# Autodesk Inventor assembly: one_servo_test
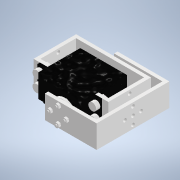
[picture p0: Inventor's stored thumbnail of the model, 180x180]
Saved by Autodesk Inventor 2021.4 (Build 254397000, 397)
## iProperties
Created: 2022-07-24
Part Number: one_servo_test
Document SubType Name: Assembly
Designer: isamu
Author: isamu
## Documents named in this file (3)
- D:\personal_projects\robot\inventor\2021_export_exp\one_servo_test.iam
- D:\personal_projects\robot\inventor\2021_export_exp\mg996r_rot_frame.iam
- D:\personal_projects\robot\inventor\2021_export_exp\mg996r_servo_frame_with_axis.iam
## Components (2 placed, 2 different names)
1. mg996r_servo_frame_with_axis:1 [sub-assembly] — Mate:1, Mate:2
2. mg996r_rot_frame:1 [sub-assembly] — Mate:1, Mate:2
## Relationships (2: Mate 2)
- Mate:1: mg996r_servo_frame_with_axis:1 ↔ mg996r_rot_frame:1
- Mate:2: mg996r_servo_frame_with_axis:1 ↔ mg996r_rot_frame:1
